# Autodesk Inventor assembly: Banhxenew
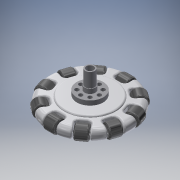
[picture p0: Inventor's stored thumbnail of the model, 180x180]
Saved by Autodesk Inventor 2019 (Build 230136000, 136)
## iProperties
Created: 2021-01-20
Part Number: Banhxenew
Document SubType Name: Assembly
Designer: Admin
Author: Admin
## Documents named in this file (3)
- C:\Users\Admin\Documents\Inventor\Doan\Banhxenew.iam
- C:\Users\Admin\Documents\Inventor\Doan\Hubnew.ipt
- C:\Users\Admin\Documents\Inventor\Doan\Omninew.ipt
## Components (2 placed, 2 different names)
1. Hubnew:1 — Mate:1, Mate:2, Mate:3
2. Omninew:1 — Mate:1, Mate:2, Mate:3
## Relationships (3: Mate 3)
- Mate:1: Hubnew:1 ↔ Omninew:1
- Mate:2: Hubnew:1 ↔ Omninew:1
- Mate:3: Hubnew:1 ↔ Omninew:1
